# Autodesk Inventor assembly: Fr.wing_assy
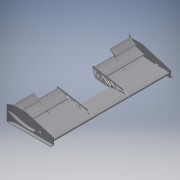
[picture p0: Inventor's stored thumbnail of the model, 180x180]
Saved by Autodesk Inventor 2018.3 (Build 223284000, 284)
## iProperties
Created: 2018-03-05
Part Number: Fr.wing_assy
Material: 一般
Document SubType Name: Assembly
Designer: ku_sk
Mass: 11232.8 g
Surface Area: 27769.7 cm^2
Volume: 11454.5 cm^3
Density: 0.980642 g/cm^3
Author: ku_sk
## Documents named in this file (15)
- D:\ku_sk\ドキュメント\Inventor\Aero\KS-15\Fr.wing\Fr.wing_assy.iam
- D:\ku_sk\ドキュメント\Inventor\Aero\KS-15\Fr.wing\parts\mainflap_side\mainflap_side.iam
- D:\ku_sk\ドキュメント\Inventor\Aero\KS-15\Fr.wing\parts\mainflap_center\mainflap_center.iam
- D:\ku_sk\ドキュメント\Inventor\Aero\KS-15\Fr.wing\parts\subflap\subflap.iam
- D:\ku_sk\ドキュメント\Inventor\Aero\KS-15\Fr.wing\parts\bracket1\bracket1.ipt
- D:\ku_sk\ドキュメント\Inventor\Aero\KS-15\Fr.wing\parts\axis_f2.ipt
- D:\ku_sk\ドキュメント\Inventor\Aero\KS-15\Fr.wing\parts\axis_f1.ipt
- D:\ku_sk\ドキュメント\Inventor\Aero\KS-15\Fr.wing\parts\gurnee.ipt
- D:\ku_sk\ドキュメント\Inventor\Aero\KS-15\Fr.wing\parts\splitter\splitter.iam
- D:\ku_sk\ドキュメント\Inventor\Aero\KS-15\Fr.wing\parts\splitter\splitter_MIR.iam
- D:\ku_sk\ドキュメント\Inventor\Aero\KS-15\Fr.wing\parts\newsubflap_top.ipt
- D:\ku_sk\ドキュメント\Inventor\Aero\KS-15\Fr.wing\parts\newbracket2.ipt
- D:\ku_sk\ドキュメント\Inventor\Aero\KS-15\Fr.wing\parts\endplate\ver.2\endplate_ver211.iam
- D:\ku_sk\ドキュメント\Inventor\Aero\KS-15\Fr.wing\parts\newsubflap_top1.ipt
- D:\ku_sk\ドキュメント\Inventor\Aero\KS-15\Fr.wing\parts\endplate\ver.2\endplate_ver2111.iam
## Components (27 placed, 14 different names)
1. mainflap_center:1 [sub-assembly] — フラッシュ:1, メイト:1, メイト:4, メイト:5, メイト:6, メイト:7, 角度:1, メイト:50, メイト:51, メイト:52, メイト:53, メイト:54, メイト:55
2. mainflap_side:1 [sub-assembly] — メイト:4, メイト:7, メイト:8, メイト:9, メイト:10, フラッシュ:2, メイト:64, メイト:110
3. mainflap_side:2 [sub-assembly] — メイト:5, メイト:6, メイト:11, メイト:12, メイト:13, フラッシュ:4, メイト:65, メイト:93, メイト:107
4. mainflap_side:3 [sub-assembly] — メイト:8, メイト:9, メイト:10, フラッシュ:3, メイト:78, メイト:79, フラッシュ:20
5. mainflap_side:4 [sub-assembly] — メイト:11, メイト:12, メイト:13, フラッシュ:5
6. subflap:1 [sub-assembly] — メイト:14, メイト:15, メイト:19, フラッシュ:2, メイト:20, メイト:21
7. subflap:2 [sub-assembly] — メイト:14, メイト:15, メイト:19, フラッシュ:3
8. subflap:4 [sub-assembly] — メイト:16, メイト:17, メイト:18, フラッシュ:4, メイト:20, メイト:21, メイト:87, 正接:1, 正接:2
9. subflap:5 [sub-assembly] — メイト:16, メイト:17, メイト:18, フラッシュ:5, メイト:76, フラッシュ:18, メイト:77
10. bracket1:1 — メイト:52, メイト:53, メイト:54, メイト:65, メイト:88
11. bracket1:2 — メイト:50, メイト:51, メイト:55, メイト:64, メイト:74, メイト:75, フラッシュ:16, メイト:89
12. axis_f2:1 — フラッシュ:17, メイト:77
13. axis_f2:2 — フラッシュ:17, メイト:76, フラッシュ:18
14. axis_f2:3 — フラッシュ:15, メイト:75, フラッシュ:16
15. axis_f2:4 — フラッシュ:15, メイト:74
16. axis_f1:1 — フラッシュ:19, メイト:79
17. axis_f1:2 — フラッシュ:19, メイト:78, フラッシュ:20
18. gurnee:1 — メイト:87, 正接:1, 正接:2, メイト:88, フラッシュ:26, フラッシュ:27
19. gurnee:2 — フラッシュ:26, フラッシュ:27, メイト:89
20. splitter:2 [sub-assembly] — メイト:93
21. splitter_MIR:1 [sub-assembly]
22. newsubflap_top:1
23. newbracket2:1 — メイト:108, メイト:109, メイト:110
24. newbracket2:2 — メイト:105, メイト:106, メイト:107
25. endplate_ver211:1 [sub-assembly] — メイト:105, メイト:106, メイト:108, メイト:109
26. newsubflap_top1:1
27. endplate_ver2111:1 [sub-assembly]
## Relationships (59: Mate 43, Flush 13, Tangent 2, Angle 1)
- フラッシュ:1 [Flush]: mainflap_center:1
- メイト:1 [Mate]: mainflap_center:1
- メイト:4 [Mate]: mainflap_center:1 ↔ mainflap_side:1
- メイト:5 [Mate]: mainflap_center:1 ↔ mainflap_side:2
- メイト:6 [Mate]: mainflap_center:1 ↔ mainflap_side:2
- メイト:7 [Mate]: mainflap_center:1 ↔ mainflap_side:1
- メイト:8 [Mate] (4 mm): mainflap_side:1 ↔ mainflap_side:3
- メイト:9 [Mate]: mainflap_side:1 ↔ mainflap_side:3
- メイト:10 [Mate]: mainflap_side:1 ↔ mainflap_side:3
- メイト:11 [Mate] (4 mm): mainflap_side:2 ↔ mainflap_side:4
- メイト:12 [Mate]: mainflap_side:2 ↔ mainflap_side:4
- メイト:13 [Mate]: mainflap_side:2 ↔ mainflap_side:4
- メイト:14 [Mate]: subflap:1 ↔ subflap:2
- メイト:15 [Mate]: subflap:1 ↔ subflap:2
- メイト:16 [Mate] (4 mm): subflap:4 ↔ subflap:5
- メイト:17 [Mate]: subflap:4 ↔ subflap:5
- メイト:18 [Mate]: subflap:4 ↔ subflap:5
- メイト:19 [Mate] (4 mm): subflap:1 ↔ subflap:2
- フラッシュ:2 [Flush]: mainflap_side:1 ↔ subflap:1
- フラッシュ:3 [Flush]: mainflap_side:3 ↔ subflap:2
- フラッシュ:4 [Flush]: mainflap_side:2 ↔ subflap:4
- フラッシュ:5 [Flush]: mainflap_side:4 ↔ subflap:5
- メイト:20 [Mate]: subflap:1 ↔ subflap:4
- メイト:21 [Mate]: subflap:1 ↔ subflap:4
- 角度:1 [Angle] (4 deg): mainflap_center:1
- メイト:50 [Mate]: mainflap_center:1 ↔ bracket1:2
- メイト:51 [Mate]: mainflap_center:1 ↔ bracket1:2
- メイト:52 [Mate]: mainflap_center:1 ↔ bracket1:1
- メイト:53 [Mate]: mainflap_center:1 ↔ bracket1:1
- メイト:54 [Mate]: mainflap_center:1 ↔ bracket1:1
- メイト:55 [Mate]: mainflap_center:1 ↔ bracket1:2
- メイト:64 [Mate]: mainflap_side:1 ↔ bracket1:2
- メイト:65 [Mate]: mainflap_side:2 ↔ bracket1:1
- フラッシュ:15 [Flush]: axis_f2:3 ↔ axis_f2:4
- メイト:74 [Mate]: bracket1:2 ↔ axis_f2:4
- メイト:75 [Mate]: bracket1:2 ↔ axis_f2:3
- フラッシュ:16 [Flush]: bracket1:2 ↔ axis_f2:3
- フラッシュ:17 [Flush]: axis_f2:1 ↔ axis_f2:2
- メイト:76 [Mate]: subflap:5 ↔ axis_f2:2
- フラッシュ:18 [Flush]: subflap:5 ↔ axis_f2:2
- メイト:77 [Mate]: subflap:5 ↔ axis_f2:1
- フラッシュ:19 [Flush]: axis_f1:1 ↔ axis_f1:2
- メイト:78 [Mate]: mainflap_side:3 ↔ axis_f1:2
- メイト:79 [Mate]: mainflap_side:3 ↔ axis_f1:1
- フラッシュ:20 [Flush]: mainflap_side:3 ↔ axis_f1:2
- メイト:87 [Mate]: subflap:4 ↔ gurnee:1
- 正接:1 [Tangent]: subflap:4 ↔ gurnee:1
- 正接:2 [Tangent]: subflap:4 ↔ gurnee:1
- メイト:88 [Mate]: bracket1:1 ↔ gurnee:1
- フラッシュ:26 [Flush]: gurnee:1 ↔ gurnee:2
- フラッシュ:27 [Flush]: gurnee:1 ↔ gurnee:2
- メイト:89 [Mate]: bracket1:2 ↔ gurnee:2
- メイト:93 [Mate]: mainflap_side:2 ↔ splitter:2
- メイト:105 [Mate]: newbracket2:2 ↔ endplate_ver211:1
- メイト:106 [Mate]: newbracket2:2 ↔ endplate_ver211:1
- メイト:107 [Mate]: mainflap_side:2 ↔ newbracket2:2
- メイト:108 [Mate]: newbracket2:1 ↔ endplate_ver211:1
- メイト:109 [Mate]: newbracket2:1 ↔ endplate_ver211:1
- メイト:110 [Mate]: mainflap_side:1 ↔ newbracket2:1
